# Autodesk Inventor assembly: шутер
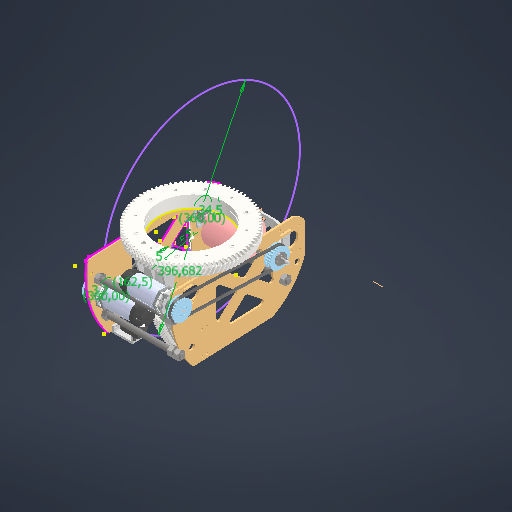
[picture p0: Inventor's stored thumbnail of the model, 512x512]
Saved by Autodesk Inventor 2026.2 (Build 302298000, 298)
## iProperties
Created: 2026-01-10
Part Number: шутер
Document SubType Name: Assembly
Designer: GameHD
Author: GameHD
## Documents named in this file (28)
- C:\Users\Phantom\Desktop\Phantom16950\шутер.iam
- C:\Users\Phantom\Desktop\Phantom16950\стенка пуляло.ipt
- C:\Users\Phantom\Desktop\Phantom16950\шевронное очко.iam
- C:\Users\Phantom\Desktop\Phantom16950\шестерня стрелять\шестерня стрелять\шестерня стрелять.ipt
- C:\Users\Phantom\Desktop\Phantom16950\изгиб новый.ipt
- C:\Users\Phantom\Desktop\Phantom16950\СИСЬКА.ipt
- C:\Users\Phantom\Desktop\Phantom16950\угол 25-26_MIR_MIR.ipt
- C:\Users\Phantom\Desktop\Phantom16950\серва мотор.ipt
- C:\Users\Phantom\Desktop\Phantom16950\шестерни прямые изменяемая траектория.iam
- C:\Users\Phantom\Desktop\Phantom16950\крепл сервы на пуляло.ipt
- C:\Users\GameHD\Downloads\Telegram Desktop\шестерня прям мал для траектории (2)\шестерня прям мал для траектории (2)\шестерня прям мал для траектории (2).ipt
- C:\Users\Phantom\Desktop\Phantom16950\стенка пуляло ответная.ipt
- C:\Users\Phantom\Desktop\Phantom16950\REV-41-1600\REV-41-1600.iam
- C:\Users\Phantom\Desktop\Phantom16950\вал 25-26.ipt
- C:\Users\Phantom\Desktop\Phantom16950\внутр сиськи.ipt
- C:\Users\Phantom\Desktop\Phantom16950\шкив 10мм\шкив 10мм\шкив 10мм.ipt
- C:\Users\Phantom\Desktop\Phantom16950\шкив прямая передача ВИКТОР ОБОСРАЛСЯ\шкив прямая передача ВИКТОР ОБОСРАЛСЯ\шкив прямая передача ВИКТОР ОБОСРАЛСЯ.ipt
- C:\Users\Phantom\Desktop\Phantom16950\для подшипника 25-26.ipt
- C:\Users\Phantom\Desktop\Phantom16950\BS 290 SKF - SKF 626-RZ.ipt
- C:\Users\Phantom\Desktop\Phantom16950\МУФТА НА ВАЛ.ipt
- C:\Users\Phantom\Desktop\Phantom16950\шкив 10мм\шкив 10мм\шкив 10мм_MIR.ipt
- C:\Users\Phantom\Desktop\Phantom16950\шкив прямая передача ВИКТОР ОБОСРАЛСЯ\шкив прямая передача ВИКТОР ОБОСРАЛСЯ\шкив прямая передача ВИКТОР ОБОСРАЛСЯ_MIR.ipt
- C:\Users\Phantom\Desktop\Phantom16950\шутер\Мастер проектирования\Передача клиновым ремнем1.iam
- C:\Users\Phantom\Desktop\Phantom16950\шутер\Мастер проектирования\Передача клиновым ремнем1_MIR.iam
- C:\Users\Phantom\Desktop\Phantom16950\ISO 4032 - M10BS EN.ipt
- C:\Users\Phantom\Desktop\Phantom16950\DIN 976-1 - M10 x 170 - A.ipt
- C:\Users\Phantom\Desktop\Phantom16950\МУФТА НА ВАЛ бол.ipt
- C:\Users\Phantom\Desktop\Phantom16950\распорка шутера 1.ipt
## Components (48 placed, 27 different names)
1. стенка пуляло:1 — Совмещение:5, Совмещение:98, Заподлицо:7
2. шевронное очко:1 [sub-assembly]
3. шестерня стрелять:1 — Совмещение:5, Совмещение:7, Совмещение:31, Совмещение:32, Совмещение:37, Совмещение:98, Совмещение:99
4. изгиб новый:1 — Заподлицо:2, Совмещение:10, Совмещение:25
5. СИСЬКА:1 — Совмещение:6, Заподлицо:2, Вставка:1, Совмещение:56
6. угол 25-26_MIR_MIR:1 — Совмещение:7
7. серва мотор:1 — Совмещение:18, Совмещение:19, Совмещение:21, Совмещение:22, Совмещение:23, Совмещение:24
8. шестерни прямые изменяемая траектория:1 [sub-assembly] — Совмещение:10, Совмещение:25, ЗубчПер:1
9. крепл сервы на пуляло:1 — Заподлицо:3, Совмещение:18, Совмещение:19
10. крепл сервы на пуляло:2 — Заподлицо:3, Совмещение:21, Совмещение:23
11. шестерня прям мал для траектории (2):1 — Совмещение:22, Совмещение:24, ЗубчПер:1
12. стенка пуляло ответная:1 — Заподлицо:7, Совмещение:99
13. угол 25-26_MIR_MIR:2 — Совмещение:31, Совмещение:32
14. REV-41-1600:1 [sub-assembly] — Совмещение:38, Совмещение:39
15. REV-41-1600:2 [sub-assembly] — Совмещение:57, Совмещение:58
16. вал 25-26:1 — Совмещение:41, Совмещение:42, Совмещение:48, Совмещение:49, Совмещение:52, Совмещение:54, Совмещение:59, Совмещение:88, Совмещение:91, Совмещение:93
17. внутр сиськи:1 — Вставка:1, Совмещение:41, Совмещение:56, Совмещение:92
18. шкив 10мм:1 — Заподлицо:4, Заподлицо:6, Совмещение:89
19. шкив прямая передача ВИКТОР ОБОСРАЛСЯ:1 — Совмещение:38, Совмещение:39, Заподлицо:4
20. для подшипника 25-26:2 — Совмещение:42, Совмещение:50, Совмещение:6
21. для подшипника 25-26:3 — Совмещение:51
22. BS 290 SKF - SKF 626-RZ:1 — Совмещение:48, Совмещение:50, Совмещение:53
23. BS 290 SKF - SKF 626-RZ:2 — Совмещение:49, Совмещение:51, Совмещение:55
24. МУФТА НА ВАЛ:1 — Совмещение:52, Совмещение:53
25. МУФТА НА ВАЛ:2 — Совмещение:54, Совмещение:55
26. шкив 10мм_MIR:1 — Заподлицо:5, Совмещение:90
27. шкив прямая передача ВИКТОР ОБОСРАЛСЯ_MIR:1 — Заподлицо:5, Совмещение:57, Совмещение:58, Совмещение:60
28. Передача клиновым ремнем:1 [sub-assembly] — Совмещение:59, Заподлицо:6
29. Передача клиновым ремнем1_MIR:1 [sub-assembly] — Совмещение:60
30. BS EN 24032 - метрическая M10:1
31. BS EN 24032 - метрическая M10:2
32. BS EN 24032 - метрическая M10:3
33. BS EN 24032 - метрическая M10:4
34. DIN 976-1 A M10 x 170:1
35. BS EN 24032 - метрическая M10:5
36. BS EN 24032 - метрическая M10:6
37. BS EN 24032 - метрическая M10:7
38. BS EN 24032 - метрическая M10:8
39. DIN 976-1 A M10 x 170:2
40. BS EN 24032 - метрическая M10:9
41. BS EN 24032 - метрическая M10:10
42. BS EN 24032 - метрическая M10:11
43. BS EN 24032 - метрическая M10:12
44. DIN 976-1 A M10 x 170:3
45. МУФТА НА ВАЛ:3 — Совмещение:90, Совмещение:91
46. МУФТА НА ВАЛ:4 — Совмещение:88, Совмещение:89
47. МУФТА НА ВАЛ бол:1 — Совмещение:92, Совмещение:93
48. распорка шутера 1:1
## Relationships (64: Mate 55, Flush 7, RelateRotation 1, Insert 1)
- [Flush]: шевронное очко:1 ↔ шестерня стрелять:1
- [Mate]: шевронное очко:1 ↔ шестерня стрелять:1
- [Mate]: шестерня стрелять:1 ↔ изгиб новый:1
- [Mate]: шестерня стрелять:1 ↔ изгиб новый:1
- [Mate]: шестерня стрелять:1 ↔ изгиб новый:1
- Совмещение:5 [Mate]: стенка пуляло:1 ↔ шестерня стрелять:1
- Совмещение:6 [Mate]: СИСЬКА:1 ↔ для подшипника 25-26:2
- Совмещение:7 [Mate]: шестерня стрелять:1 ↔ угол 25-26_MIR_MIR:1
- Заподлицо:2 [Flush]: изгиб новый:1 ↔ СИСЬКА:1
- Совмещение:10 [Mate]: изгиб новый:1 ↔ шестерни прямые изменяемая траектория:1
- Заподлицо:3 [Flush]: крепл сервы на пуляло:1 ↔ крепл сервы на пуляло:2
- Совмещение:18 [Mate]: серва мотор:1 ↔ крепл сервы на пуляло:1
- Совмещение:19 [Mate]: серва мотор:1 ↔ крепл сервы на пуляло:1
- Совмещение:21 [Mate]: серва мотор:1 ↔ крепл сервы на пуляло:2
- Совмещение:22 [Mate] (3.5 mm): серва мотор:1 ↔ шестерня прям мал для траектории (2):1
- Совмещение:23 [Mate]: серва мотор:1 ↔ крепл сервы на пуляло:2
- Совмещение:24 [Mate]: серва мотор:1 ↔ шестерня прям мал для траектории (2):1
- Совмещение:25 [Mate]: изгиб новый:1 ↔ шестерни прямые изменяемая траектория:1
- ЗубчПер:1 [RelateRotation] (0.933 ul): шестерни прямые изменяемая траектория:1 ↔ шестерня прям мал для траектории (2):1
- Совмещение:31 [Mate]: шестерня стрелять:1 ↔ угол 25-26_MIR_MIR:2
- Совмещение:32 [Mate]: шестерня стрелять:1 ↔ угол 25-26_MIR_MIR:2
- Совмещение:37 [Mate]: шестерня стрелять:1
- Совмещение:38 [Mate]: REV-41-1600:1 ↔ шкив прямая передача ВИКТОР ОБОСРАЛСЯ:1
- Совмещение:39 [Mate]: REV-41-1600:1 ↔ шкив прямая передача ВИКТОР ОБОСРАЛСЯ:1
- Заподлицо:4 [Flush]: шкив 10мм:1 ↔ шкив прямая передача ВИКТОР ОБОСРАЛСЯ:1
- Вставка:1 [Insert]: СИСЬКА:1 ↔ внутр сиськи:1
- Совмещение:41 [Mate]: вал 25-26:1 ↔ внутр сиськи:1
- Совмещение:42 [Mate]: вал 25-26:1 ↔ для подшипника 25-26:2
- Совмещение:48 [Mate]: вал 25-26:1 ↔ BS 290 SKF - SKF 626-RZ:1
- Совмещение:49 [Mate]: вал 25-26:1 ↔ BS 290 SKF - SKF 626-RZ:2
- Совмещение:50 [Mate]: для подшипника 25-26:2 ↔ BS 290 SKF - SKF 626-RZ:1
- Совмещение:51 [Mate]: для подшипника 25-26:3 ↔ BS 290 SKF - SKF 626-RZ:2
- Совмещение:52 [Mate]: вал 25-26:1 ↔ МУФТА НА ВАЛ:1
- Совмещение:53 [Mate]: BS 290 SKF - SKF 626-RZ:1 ↔ МУФТА НА ВАЛ:1
- Совмещение:54 [Mate]: вал 25-26:1 ↔ МУФТА НА ВАЛ:2
- Совмещение:55 [Mate]: BS 290 SKF - SKF 626-RZ:2 ↔ МУФТА НА ВАЛ:2
- Совмещение:56 [Mate]: СИСЬКА:1 ↔ внутр сиськи:1
- Заподлицо:5 [Flush]: шкив 10мм_MIR:1 ↔ шкив прямая передача ВИКТОР ОБОСРАЛСЯ_MIR:1
- Совмещение:57 [Mate]: REV-41-1600:2 ↔ шкив прямая передача ВИКТОР ОБОСРАЛСЯ_MIR:1
- Совмещение:58 [Mate]: REV-41-1600:2 ↔ шкив прямая передача ВИКТОР ОБОСРАЛСЯ_MIR:1
- Совмещение:59 [Mate]: вал 25-26:1 ↔ Передача клиновым ремнем:1
- Заподлицо:6 [Flush] (1.5 mm): шкив 10мм:1 ↔ Передача клиновым ремнем:1
- Совмещение:60 [Mate]: шкив прямая передача ВИКТОР ОБОСРАЛСЯ_MIR:1 ↔ Передача клиновым ремнем1_MIR:1
- [Mate]: BS EN 24032 - метрическая M10:3 ↔ DIN 976-1 A M10 x 170:1
- [Mate]: BS EN 24032 - метрическая M10:1 ↔ DIN 976-1 A M10 x 170:1
- [Mate]: BS EN 24032 - метрическая M10:4 ↔ DIN 976-1 A M10 x 170:1
- [Mate]: BS EN 24032 - метрическая M10:2 ↔ DIN 976-1 A M10 x 170:1
- [Mate]: BS EN 24032 - метрическая M10:7 ↔ DIN 976-1 A M10 x 170:2
- [Mate]: BS EN 24032 - метрическая M10:5 ↔ DIN 976-1 A M10 x 170:2
- [Mate]: BS EN 24032 - метрическая M10:8 ↔ DIN 976-1 A M10 x 170:2
- [Mate]: BS EN 24032 - метрическая M10:6 ↔ DIN 976-1 A M10 x 170:2
- [Mate]: BS EN 24032 - метрическая M10:11 ↔ DIN 976-1 A M10 x 170:3
- [Mate]: BS EN 24032 - метрическая M10:9 ↔ DIN 976-1 A M10 x 170:3
- [Mate]: BS EN 24032 - метрическая M10:12 ↔ DIN 976-1 A M10 x 170:3
- [Mate]: BS EN 24032 - метрическая M10:10 ↔ DIN 976-1 A M10 x 170:3
- Совмещение:88 [Mate]: вал 25-26:1 ↔ МУФТА НА ВАЛ:4
- Совмещение:89 [Mate]: шкив 10мм:1 ↔ МУФТА НА ВАЛ:4
- Совмещение:90 [Mate]: шкив 10мм_MIR:1 ↔ МУФТА НА ВАЛ:3
- Совмещение:91 [Mate]: вал 25-26:1 ↔ МУФТА НА ВАЛ:3
- Совмещение:92 [Mate]: внутр сиськи:1 ↔ МУФТА НА ВАЛ бол:1
- Совмещение:93 [Mate]: вал 25-26:1 ↔ МУФТА НА ВАЛ бол:1
- Совмещение:98 [Mate] (29 mm): стенка пуляло:1 ↔ шестерня стрелять:1
- Заподлицо:7 [Flush]: стенка пуляло:1 ↔ стенка пуляло ответная:1
- Совмещение:99 [Mate] (29 mm): шестерня стрелять:1 ↔ стенка пуляло ответная:1
## Named parameters: d93_d66 = 0 mm, d94_d67 = 0 mm, d95_d68 = 0 mm, d96_d69 = 0 mm, d75_d66 = 0 mm, d76_d67 = 0 mm, d77_d68 = 0 mm, d78_d69 = 0 mm, d79_d66 = 0 mm, d80_d67 = 0 mm, d81_d68 = 0 mm, d82_d69 = 0 mm
